# Autodesk Inventor assembly: x-axis
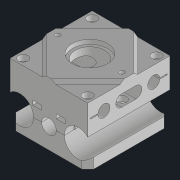
[picture p0: Inventor's stored thumbnail of the model, 180x180]
Saved by Autodesk Inventor 2021 (Build 250183000, 183)
## iProperties
Created: 2021-06-07
Part Number: x-axis
Document SubType Name: Assembly
Designer: arbra
Author: arbra
## Documents named in this file (3)
- C:\Users\arbra\OneDrive\Documents\3D Printer\IPT\ASSEMBLY\x-axis.iam
- C:\Users\arbra\OneDrive\Documents\3D Printer\IPT\PARTS\Z-AXIS\z-carriage-front.ipt
- C:\Users\arbra\OneDrive\Documents\3D Printer\IPT\PARTS\Z-AXIS\z-carriage-rear.ipt
## Components (2 placed, 2 different names)
1. z-carriage-front:1 — Mate:1, Insert:1, Insert:2
2. z-carriage-rear:1 — Mate:1, Insert:1, Insert:2
## Relationships (3: Insert 2, Mate 1)
- Mate:1: z-carriage-front:1 ↔ z-carriage-rear:1
- Insert:1: z-carriage-front:1 ↔ z-carriage-rear:1
- Insert:2: z-carriage-front:1 ↔ z-carriage-rear:1
